# Autodesk Inventor assembly: BackMountAssembly_SimplfiedVersion
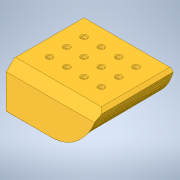
[picture p0: Inventor's stored thumbnail of the model, 180x180]
Saved by Autodesk Inventor 2021 (Build 250183000, 183)
## iProperties
Created: 2019-05-05
Part Number: BackMountAssembly_SimplfiedVersion
Document SubType Name: Assembly
Designer: lgnds
Author: lgnds
## Documents named in this file (2)
- C:\Users\Viktor\Google Drive\Chalmers\Fortsatt arbete WR\Design files\FRS - Front Rail System_V2\FästenFörRam\BackMountAssembly_SimplfiedVersion.iam
- C:\Users\Viktor\Google Drive\Chalmers\Fortsatt arbete WR\Design files\FRS - Front Rail System_V2\FästenFörRam\BakV4_SimplifiedVersionV2.ipt
## Components (1 placed, 1 different names)
1. BakV4_SimplifiedVersionV2:1 — Mate:1, Flush:1, Flush:2
## Relationships (3: Flush 2, Mate 1)
- Mate:1 (183 mm): BakV4_SimplifiedVersionV2:1
- Flush:1 (58 mm): BakV4_SimplifiedVersionV2:1
- Flush:2 (-45 mm): BakV4_SimplifiedVersionV2:1
